# Autodesk Inventor assembly: Assembly
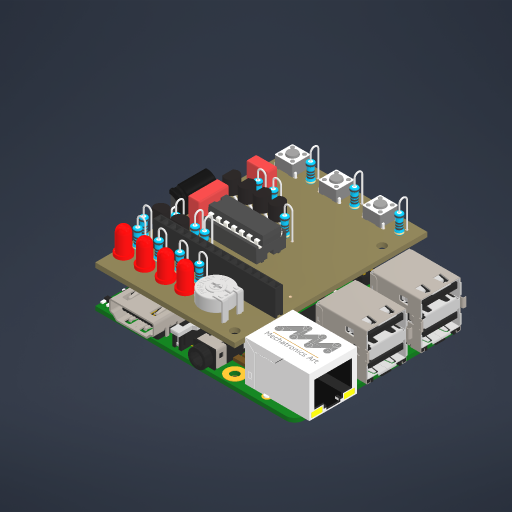
[picture p0: Inventor's stored thumbnail of the model, 512x512]
Saved by Autodesk Inventor 2023 (Build 270158000, 158)
## iProperties
Created: 2022-12-07
Part Number: Assembly
Document SubType Name: Assembly
Designer: Manuel
Author: Manuel
## Documents named in this file (3)
- C:\workspace\Studium\WST\opcua_netzwerk\Entwicklung Knoten\3D Modell\Assembly.iam
- C:\workspace\Studium\WST\opcua_netzwerk\Entwicklung Knoten\3D Modell\ConnectorHead_RPi\ConnectorHead_RPi.iam
- C:\workspace\Studium\WST\opcua_netzwerk\Entwicklung Knoten\3D Modell\Raspberry Pi 3B\Raspberry Pi 3.iam
## Components (2 placed, 2 different names)
1. Raspberry Pi 3:1 [sub-assembly] — Fluchtend:1, Fluchtend:2, Passend:1
2. ConnectorHead_RPi:1 [sub-assembly] — Fluchtend:1, Fluchtend:2, Passend:1
## Relationships (3: Flush 2, Mate 1)
- Fluchtend:1 [Flush]: Raspberry Pi 3:1 ↔ ConnectorHead_RPi:1
- Fluchtend:2 [Flush]: Raspberry Pi 3:1 ↔ ConnectorHead_RPi:1
- Passend:1 [Mate] (11 mm): Raspberry Pi 3:1 ↔ ConnectorHead_RPi:1
